# Autodesk Inventor assembly: rec
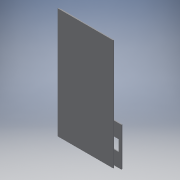
[picture p0: Inventor's stored thumbnail of the model, 180x180]
Saved by Autodesk Inventor 2019 (Build 230136000, 136)
## iProperties
Created: 2021-11-18
Part Number: rec
Material: 一般
Document SubType Name: Assembly
Designer: yuta
Author: yuta
## Documents named in this file (4)
- C:\Users\yuta\Documents\キャチロボ\rec.iam
- C:\Users\yuta\Documents\キャチロボ\NC.port.ipt
- C:\Users\yuta\Documents\キャチロボ\came1.ipt
- C:\Users\yuta\Documents\キャチロボ\came2.ipt
## Components (6 placed, 3 different names)
1. NC.port:1 — メイト:1, フラッシュ:1, メイト:2, メイト:3, メイト:4, メイト:5
2. came1:1 — メイト:1, フラッシュ:1
3. came1:2 — メイト:2
4. came2:1 — メイト:3
5. came2:2 — メイト:4
6. came2:3 — メイト:5
## Relationships (6: Mate 5, Flush 1)
- メイト:1 [Mate]: NC.port:1 ↔ came1:1
- フラッシュ:1 [Flush] (6 mm): NC.port:1 ↔ came1:1
- メイト:2 [Mate]: NC.port:1 ↔ came1:2
- メイト:3 [Mate]: NC.port:1 ↔ came2:1
- メイト:4 [Mate]: NC.port:1 ↔ came2:2
- メイト:5 [Mate]: NC.port:1 ↔ came2:3
